# Autodesk Inventor assembly: 組合檔
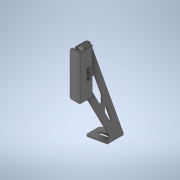
[picture p0: Inventor's stored thumbnail of the model, 180x180]
Saved by Autodesk Inventor 2020 (Build 240168000, 168)
## iProperties
Created: 2015-11-28
Part Number: 組合檔
Document SubType Name: Assembly
Designer: 設計製圖
Author: 設計製圖
## Documents named in this file (15)
- D:\資料庫\設計-3D Project\【May club 】\得利卡-車頂燈架\模型、圖面\吊架-長(R)(#11.26)\長-車頂燈架-組合(#11.26).iam
- D:\資料庫\設計-3D Project\【May club 】\得利卡-車頂燈架\模型、圖面\現成品-組裝零件\概-膠條.ipt
- D:\資料庫\設計-3D Project\【May club 】\得利卡-車頂燈架\模型、圖面\現成品-組裝零件\概-泡棉墊(3).ipt
- D:\資料庫\設計-3D Project\【 鐵蹄 】\------鐵蹄工廠素材------ -\拉帽-M8.ipt
- D:\資料庫\設計-3D Project\【May club 】\得利卡-車頂燈架\模型、圖面\焊接組件-1(#11.02).ipt
- D:\資料庫\設計-3D Project\材料庫\【螺絲】\止付螺絲\止付螺絲-M8-20.ipt
- D:\資料庫\設計-3D Project\【May club 】\得利卡-車頂燈架\模型、圖面\車身圖.ipt
- D:\資料庫\設計-3D Project\【May club 】\得利卡-車頂燈架\模型、圖面\吊架組件-ㄇ槽(#11.02).ipt
- D:\資料庫\設計-3D Project\【May club 】\得利卡-車頂燈架\模型、圖面\焊接組件-2(#11.02).ipt
- D:\資料庫\設計-3D Project\材料庫\【螺絲】\外六角螺絲\白鐵-外六角  M6-10.ipt
- D:\資料庫\設計-3D Project\【May club 】\得利卡-車頂燈架\模型、圖面\得利卡-車頂導水槽.ipt
- D:\資料庫\設計-3D Project\材料庫\螺帽\白鐵-六角螺帽-M6.ipt
- D:\資料庫\設計-3D Project\【May club 】\得利卡-車頂燈架\模型、圖面\現成品-組裝零件\概-泡棉墊2.5t(1).ipt
- D:\資料庫\設計-3D Project\【May club 】\得利卡-車頂燈架\模型、圖面\現成品-組裝零件\概-泡棉墊6.0t(2).ipt
- D:\資料庫\設計-3D Project\【May club 】\得利卡-車頂燈架\模型、圖面\吊架-長(R)(#11.26)\吊架-長(R)(#11.26).ipt
## Components (16 placed, 14 different names)
1. 車身圖:1 — 貼合:33
2. 得利卡-車頂導水槽:1 — 角度:1, 齊平:17
3. 吊架組件-ㄇ槽(#11.02):1 — 貼合:6, 齊平:2, 齊平:3, 貼合:8, 齊平:4, 貼合:17, 貼合:35, 貼合:36, 貼合:37, 貼合:38, 貼合:40, 齊平:14, 貼合:41, 貼合:18, 齊平:13, 齊平:16
4. 吊架-長(R)(#11.26):1 — 貼合:3, 貼合:4, 齊平:1, 貼合:18, 貼合:23, 貼合:25, 貼合:26, 貼合:33, 貼合:43, 齊平:18
5. 焊接組件-1(#11.02):1 — 貼合:23, 貼合:25, 貼合:26, 貼合:27, 齊平:7, 齊平:8, 齊平:13, 齊平:16
6. 拉帽-M8:1 — 齊平:6, 貼合:15, 貼合:17, 貼合:31, 貼合:35, 貼合:37
7. 拉帽-M8:2 — 齊平:6, 貼合:15, 貼合:32, 貼合:36, 貼合:38
8. 焊接組件-2(#11.02):1 — 貼合:40, 齊平:14, 貼合:41, 貼合:44, 貼合:45, 齊平:15
9. 白鐵-外六角  M6-10:1 — 貼合:43, 貼合:46
10. 白鐵-六角螺帽-M6:1 — 貼合:44, 貼合:45, 齊平:15, 貼合:46
11. 概-泡棉墊6.0t(2):1 — 貼合:27, 齊平:7, 齊平:8
12. 概-膠條:1 — 貼合:3, 貼合:4, 齊平:1
13. 概-泡棉墊2.5t(1):1 — 貼合:6, 齊平:2, 齊平:3, 貼合:9
14. 概-泡棉墊(3):1 — 貼合:8, 貼合:9, 齊平:4
15. 止付螺絲-M8-20:1 — 齊平:12, 貼合:31
16. 止付螺絲-M8-20:2 — 齊平:12, 貼合:32
## Relationships (40: Mate 25, Flush 14, Angle 1)
- 貼合:3 [Mate]: 吊架-長(R)(#11.26):1 ↔ 概-膠條:1
- 貼合:4 [Mate]: 吊架-長(R)(#11.26):1 ↔ 概-膠條:1
- 齊平:1 [Flush]: 吊架-長(R)(#11.26):1 ↔ 概-膠條:1
- 貼合:6 [Mate]: 吊架組件-ㄇ槽(#11.02):1 ↔ 概-泡棉墊2.5t(1):1
- 齊平:2 [Flush]: 吊架組件-ㄇ槽(#11.02):1 ↔ 概-泡棉墊2.5t(1):1
- 齊平:3 [Flush]: 吊架組件-ㄇ槽(#11.02):1 ↔ 概-泡棉墊2.5t(1):1
- 貼合:8 [Mate]: 吊架組件-ㄇ槽(#11.02):1 ↔ 概-泡棉墊(3):1
- 貼合:9 [Mate]: 概-泡棉墊2.5t(1):1 ↔ 概-泡棉墊(3):1
- 齊平:4 [Flush]: 吊架組件-ㄇ槽(#11.02):1 ↔ 概-泡棉墊(3):1
- 齊平:6 [Flush]: 拉帽-M8:1 ↔ 拉帽-M8:2
- 貼合:15 [Mate]: 拉帽-M8:1 ↔ 拉帽-M8:2
- 貼合:17 [Mate]: 吊架組件-ㄇ槽(#11.02):1 ↔ 拉帽-M8:1
- 貼合:23 [Mate]: 吊架-長(R)(#11.26):1 ↔ 焊接組件-1(#11.02):1
- 貼合:25 [Mate]: 吊架-長(R)(#11.26):1 ↔ 焊接組件-1(#11.02):1
- 貼合:26 [Mate]: 吊架-長(R)(#11.26):1 ↔ 焊接組件-1(#11.02):1
- 貼合:27 [Mate]: 焊接組件-1(#11.02):1 ↔ 概-泡棉墊6.0t(2):1
- 齊平:7 [Flush]: 焊接組件-1(#11.02):1 ↔ 概-泡棉墊6.0t(2):1
- 齊平:8 [Flush]: 焊接組件-1(#11.02):1 ↔ 概-泡棉墊6.0t(2):1
- 齊平:12 [Flush]: 止付螺絲-M8-20:1 ↔ 止付螺絲-M8-20:2
- 貼合:31 [Mate]: 拉帽-M8:1 ↔ 止付螺絲-M8-20:1
- 貼合:32 [Mate]: 拉帽-M8:2 ↔ 止付螺絲-M8-20:2
- 貼合:33 [Mate]: 車身圖:1 ↔ 吊架-長(R)(#11.26):1
- 貼合:35 [Mate]: 吊架組件-ㄇ槽(#11.02):1 ↔ 拉帽-M8:1
- 貼合:36 [Mate]: 吊架組件-ㄇ槽(#11.02):1 ↔ 拉帽-M8:2
- 貼合:37 [Mate]: 吊架組件-ㄇ槽(#11.02):1 ↔ 拉帽-M8:1
- 貼合:38 [Mate]: 吊架組件-ㄇ槽(#11.02):1 ↔ 拉帽-M8:2
- 貼合:40 [Mate]: 吊架組件-ㄇ槽(#11.02):1 ↔ 焊接組件-2(#11.02):1
- 齊平:14 [Flush]: 吊架組件-ㄇ槽(#11.02):1 ↔ 焊接組件-2(#11.02):1
- 貼合:41 [Mate]: 吊架組件-ㄇ槽(#11.02):1 ↔ 焊接組件-2(#11.02):1
- 貼合:18 [Mate]: 吊架組件-ㄇ槽(#11.02):1 ↔ 吊架-長(R)(#11.26):1
- 齊平:13 [Flush]: 吊架組件-ㄇ槽(#11.02):1 ↔ 焊接組件-1(#11.02):1
- 貼合:43 [Mate]: 吊架-長(R)(#11.26):1 ↔ 白鐵-外六角  M6-10:1
- 貼合:44 [Mate]: 焊接組件-2(#11.02):1 ↔ 白鐵-六角螺帽-M6:1
- 貼合:45 [Mate]: 焊接組件-2(#11.02):1 ↔ 白鐵-六角螺帽-M6:1
- 齊平:15 [Flush]: 焊接組件-2(#11.02):1 ↔ 白鐵-六角螺帽-M6:1
- 貼合:46 [Mate]: 白鐵-外六角  M6-10:1 ↔ 白鐵-六角螺帽-M6:1
- 齊平:16 [Flush]: 吊架組件-ㄇ槽(#11.02):1 ↔ 焊接組件-1(#11.02):1
- 角度:1 [Angle] (180 deg): 得利卡-車頂導水槽:1
- 齊平:17 [Flush]: 得利卡-車頂導水槽:1
- 齊平:18 [Flush] (150 mm): 吊架-長(R)(#11.26):1
